# Autodesk Inventor assembly: ASM Main
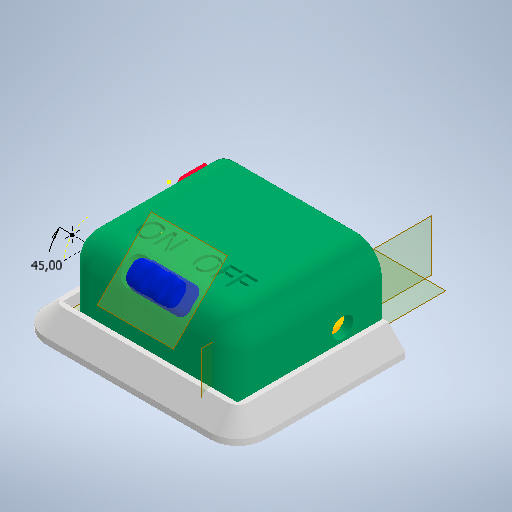
[picture p0: Inventor's stored thumbnail of the model, 512x512]
Saved by Autodesk Inventor 2025.2 (Build 292293000, 293)
## iProperties
Created: 2024-11-12
Part Number: ASM Main
Document SubType Name: Assembly
Designer: matss
Author: matss
## Documents named in this file (8)
- C:\Users\tills\Desktop\Studium\Semester_3\Repositorys\Wearable-Health-Device\ASM Main.iam
- C:\Users\tills\Desktop\Studium\Semester_3\Repositorys\Wearable-Health-Device\MCI_PCB\MCI_PCB\MCI_PCB.iam
- C:\Users\tills\Desktop\Studium\Semester_3\Repositorys\Wearable-Health-Device\PCB_Mount.ipt
- C:\Users\tills\Desktop\Studium\Semester_3\Repositorys\Wearable-Health-Device\PCB_Deckel.ipt
- C:\Users\tills\Desktop\Studium\Semester_3\Repositorys\Wearable-Health-Device\Schalter.ipt
- C:\Users\tills\Desktop\Studium\Semester_3\Repositorys\Wearable-Health-Device\Schalter_vergroeßerung.ipt
- C:\Users\tills\Desktop\Studium\Semester_3\Repositorys\Wearable-Health-Device\USB-C_cover.ipt
- C:\Users\tills\Desktop\Studium\Semester_3\Repositorys\Wearable-Health-Device\IMU_Base_T-Shirt_PCB.ipt
## Components (7 placed, 7 different names)
1. MCI_PCB:1 [sub-assembly] — Passend:4, Passend:5, Passend:6, Passend:19, Winkel:1
2. PCB_Mount:1 — Passend:1, Passend:2, Passend:3, Passend:4, Passend:5, Passend:6, Passend:7, Passend:8, Fluchtend:10, Passend:20
3. PCB_Deckel:1 — Passend:7, Passend:8, Fluchtend:10, Passend:9, Passend:10, Passend:17, Passend:18, Passend:21, Passend:22
4. Schalter:1 — Passend:12, Passend:15, Passend:16
5. Schalter_vergroeßerung:1 — Passend:9, Passend:10, Passend:12, Passend:15, Passend:16
6. USB-C_cover:1 — Passend:17, Passend:18
7. IMU_Base_T-Shirt_PCB:1 — Passend:20, Passend:21, Passend:22
## Relationships (21: Mate 19, Flush 1, Angle 1)
- Passend:1 [Mate]: PCB_Mount:1
- Passend:2 [Mate]: PCB_Mount:1
- Passend:3 [Mate] (20 mm): PCB_Mount:1
- Passend:4 [Mate] (2.5 mm): MCI_PCB:1 ↔ PCB_Mount:1
- Passend:5 [Mate]: MCI_PCB:1 ↔ PCB_Mount:1
- Passend:6 [Mate]: MCI_PCB:1 ↔ PCB_Mount:1
- Passend:7 [Mate]: PCB_Mount:1 ↔ PCB_Deckel:1
- Passend:8 [Mate]: PCB_Mount:1 ↔ PCB_Deckel:1
- Fluchtend:10 [Flush]: PCB_Mount:1 ↔ PCB_Deckel:1
- Passend:9 [Mate] (0.25 mm): PCB_Deckel:1 ↔ Schalter_vergroeßerung:1
- Passend:10 [Mate] (0.5 mm): PCB_Deckel:1 ↔ Schalter_vergroeßerung:1
- Passend:12 [Mate]: Schalter:1 ↔ Schalter_vergroeßerung:1
- Passend:15 [Mate]: Schalter:1 ↔ Schalter_vergroeßerung:1
- Passend:16 [Mate] (0.5 mm): Schalter:1 ↔ Schalter_vergroeßerung:1
- Passend:17 [Mate]: PCB_Deckel:1 ↔ USB-C_cover:1
- Passend:18 [Mate]: PCB_Deckel:1 ↔ USB-C_cover:1
- Passend:19 [Mate]: MCI_PCB:1
- Winkel:1 [Angle] (0 deg): MCI_PCB:1
- Passend:20 [Mate]: PCB_Mount:1 ↔ IMU_Base_T-Shirt_PCB:1
- Passend:21 [Mate] (0.25 mm): PCB_Deckel:1 ↔ IMU_Base_T-Shirt_PCB:1
- Passend:22 [Mate] (0.25 mm): PCB_Deckel:1 ↔ IMU_Base_T-Shirt_PCB:1
